# Autodesk Inventor assembly: Front Upper Arm
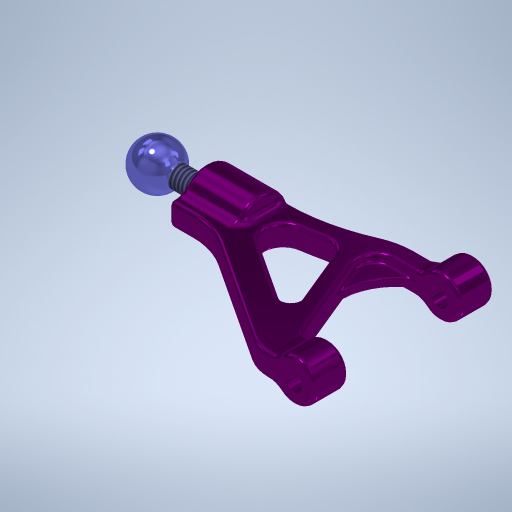
[picture p0: Inventor's stored thumbnail of the model, 512x512]
Saved by Autodesk Inventor 2023.1 (Build 271208000, 208)
## iProperties
Created: 2019-11-30
Part Number: Front Upper Arm
Document SubType Name: Assembly
Designer: Jopa
Author: Jopa
## Documents named in this file (3)
- C:\Users\Arzum Naz Doğaner\OneDrive\Masaüstü\HUDSON süspansiyon\Front Upper Arm.iam
- C:\Users\Arzum Naz Doğaner\OneDrive\Masaüstü\HUDSON süspansiyon\Front Upper Arm.ipt
- C:\Users\Arzum Naz Doğaner\OneDrive\Masaüstü\HUDSON süspansiyon\Pillow Ball.ipt
## Components (2 placed, 2 different names)
1. Front Upper Arm:1 — Mate:1, Mate:2
2. Pillow Ball:1 — Mate:1, Mate:2
## Relationships (2: Mate 2)
- Mate:1: Front Upper Arm:1 ↔ Pillow Ball:1
- Mate:2 (8.89 mm): Front Upper Arm:1 ↔ Pillow Ball:1
